# Autodesk Inventor assembly: 06_10 Plataforma
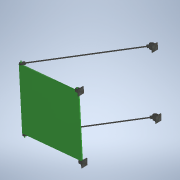
[picture p0: Inventor's stored thumbnail of the model, 180x180]
Saved by Autodesk Inventor 2021 (Build 250183000, 183)
## iProperties
Created: 2021-06-25
Part Number: 06_10 Plataforma
Document SubType Name: Assembly
Designer: Almanzor
Author: Almanzor
## Documents named in this file (12)
- C:\Users\Almanzor\Documents\Escuela\LABORATORIO DISEÑO Y MANUFACTURA ASISTIDA POR COMPUTADORA\Practica 6\06_10 Plataforma.iam
- C:\Users\Almanzor\Documents\Escuela\LABORATORIO DISEÑO Y MANUFACTURA ASISTIDA POR COMPUTADORA\Practica 6\01_10_Plataforma.ipt
- C:\Users\Almanzor\Documents\Escuela\LABORATORIO DISEÑO Y MANUFACTURA ASISTIDA POR COMPUTADORA\Practica 6\02_10 Soporte01.ipt
- C:\Users\Almanzor\Documents\Escuela\LABORATORIO DISEÑO Y MANUFACTURA ASISTIDA POR COMPUTADORA\Practica 6\03_10 soporte02.ipt
- C:\Users\Almanzor\Documents\Escuela\LABORATORIO DISEÑO Y MANUFACTURA ASISTIDA POR COMPUTADORA\Practica 6\04_10 Cable.ipt
- C:\Users\Almanzor\Documents\Escuela\LABORATORIO DISEÑO Y MANUFACTURA ASISTIDA POR COMPUTADORA\Practica 6\04_10_Birlo.ipt
- C:\Users\Almanzor\Documents\Escuela\LABORATORIO DISEÑO Y MANUFACTURA ASISTIDA POR COMPUTADORA\Practica 6\06_10 Plataforma\AIP\FEA\dnbr60e9s.fins
- C:\Users\Almanzor\Documents\Escuela\LABORATORIO DISEÑO Y MANUFACTURA ASISTIDA POR COMPUTADORA\Practica 6\06_10 Plataforma\AIP\FEA\dnbr60e9s.fsat
- C:\Users\Almanzor\Documents\Escuela\LABORATORIO DISEÑO Y MANUFACTURA ASISTIDA POR COMPUTADORA\Practica 6\06_10 Plataforma\AIP\FEA\dnbr60e9s.ftes
- C:\Users\Almanzor\Documents\Escuela\LABORATORIO DISEÑO Y MANUFACTURA ASISTIDA POR COMPUTADORA\Practica 6\06_10 Plataforma\AIP\FEA\dnbr60e9s.fwiz
- C:\Users\Almanzor\Documents\Escuela\LABORATORIO DISEÑO Y MANUFACTURA ASISTIDA POR COMPUTADORA\Practica 6\06_10 Plataforma\AIP\FEA\dnbr60ebk.fmsh
- C:\Users\Almanzor\Documents\Escuela\LABORATORIO DISEÑO Y MANUFACTURA ASISTIDA POR COMPUTADORA\Practica 6\06_10 Plataforma\AIP\FEA\dnbr60ecg.fres
## Components (9 placed, 5 different names)
1. 01_10_Plataforma:1 — De rotación:1, Cilíndrica:1, Coincidencia:1, Cilíndrica:2, Coincidencia:2, Cilíndrica:3, Coincidencia:3, Ángulo:1, Ángulo:2
2. 02_10 Soporte01:1 — Cilíndrica:2, Coincidencia:2, Ángulo:2, Nivelación:2
3. 03_10 soporte02:1 — De rotación:2, Coincidencia:4, Coincidencia:5, Nivelación:1
4. 04_10 Cable:1 — Cilíndrica:1, Coincidencia:1, De rotación:3
5. 02_10 Soporte01:2 — Cilíndrica:3, Coincidencia:3, Ángulo:1, Nivelación:1
6. 03_10 soporte02:2 — De rotación:3, Coincidencia:6, De rotación:4, Nivelación:2
7. 04_10 Cable:2 — De rotación:1, De rotación:2
8. 04_10_Birlo:1 — Coincidencia:4, Coincidencia:5
9. 04_10_Birlo:2 — Coincidencia:6, De rotación:4
## Relationships (17: Mate 6, RevoluteJoint 4, CylindricalJoint 3, Angle 2, Flush 2)
- De rotación:1 [RevoluteJoint] (-25 mm): 01_10_Plataforma:1 ↔ 04_10 Cable:2
- Cilíndrica:1 [CylindricalJoint]: 01_10_Plataforma:1 ↔ 04_10 Cable:1
- Coincidencia:1 [Mate]: 01_10_Plataforma:1 ↔ 04_10 Cable:1
- Cilíndrica:2 [CylindricalJoint]: 01_10_Plataforma:1 ↔ 02_10 Soporte01:1
- Coincidencia:2 [Mate]: 01_10_Plataforma:1 ↔ 02_10 Soporte01:1
- Cilíndrica:3 [CylindricalJoint]: 01_10_Plataforma:1 ↔ 02_10 Soporte01:2
- Coincidencia:3 [Mate]: 01_10_Plataforma:1 ↔ 02_10 Soporte01:2
- De rotación:2 [RevoluteJoint]: 03_10 soporte02:1 ↔ 04_10 Cable:2
- Coincidencia:4 [Mate]: 03_10 soporte02:1 ↔ 04_10_Birlo:1
- Coincidencia:5 [Mate]: 03_10 soporte02:1 ↔ 04_10_Birlo:1
- De rotación:3 [RevoluteJoint]: 04_10 Cable:1 ↔ 03_10 soporte02:2
- Coincidencia:6 [Mate]: 03_10 soporte02:2 ↔ 04_10_Birlo:2
- De rotación:4 [RevoluteJoint]: 03_10 soporte02:2 ↔ 04_10_Birlo:2
- Ángulo:1 [Angle] (270 deg): 01_10_Plataforma:1 ↔ 02_10 Soporte01:2
- Nivelación:1 [Flush]: 03_10 soporte02:1 ↔ 02_10 Soporte01:2
- Ángulo:2 [Angle] (90 deg): 01_10_Plataforma:1 ↔ 02_10 Soporte01:1
- Nivelación:2 [Flush]: 02_10 Soporte01:1 ↔ 03_10 soporte02:2
## Named parameters: sa_0 = 1.962e+06
note: some values were not read from the file. Shown as the stored number, unit unknown: "sa_0".
